# Autodesk Inventor assembly: GGC
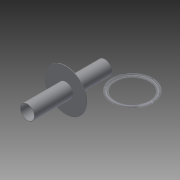
[picture p0: Inventor's stored thumbnail of the model, 180x180]
Saved by Autodesk Inventor 2015 (Build 190159000, 159)
## iProperties
Created: 2016-04-11
Part Number: GGC
Document SubType Name: Assembly
Designer: rubenjm
Author: rubenjm
## Documents named in this file (4)
- C:\Users\rubenjm\Documents\To Transfer\2k16 Spring\RME\GGC\GGC.iam
- C:\Users\rubenjm\Documents\To Transfer\2k16 Spring\RME\GGC\Turntable.ipt
- C:\Users\rubenjm\Documents\To Transfer\2k16 Spring\RME\GGC\Inner Pole.ipt
- C:\Users\rubenjm\Documents\To Transfer\2k16 Spring\RME\GGC\Base Plate.ipt
## Components (3 placed, 3 different names)
1. Turntable:1
2. Inner Pole:1 — Flush:1
3. Base Plate:1 — Flush:1
## Relationships (1: Flush 1)
- Flush:1 (304.8 mm): Inner Pole:1 ↔ Base Plate:1
